# Autodesk Inventor assembly: BoronHead
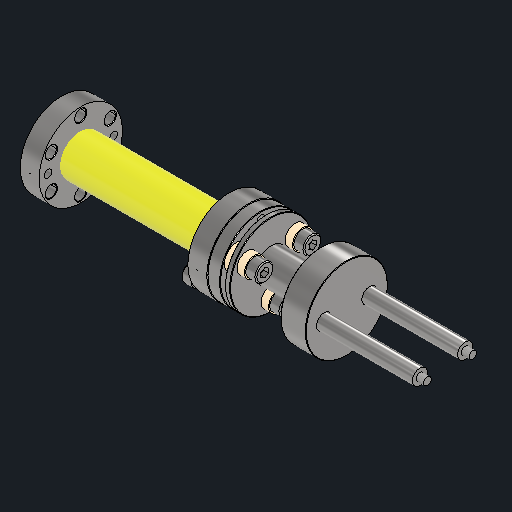
[picture p0: Inventor's stored thumbnail of the model, 512x512]
Saved by Autodesk Inventor 2027.1 (Build 311270010, 270A)
## iProperties
Created: 2025-06-19
Part Number: BoronHead
Document SubType Name: Assembly
Designer: kuzmin
Author: kuzmin
## Documents named in this file (8)
- C:\Users\queezz\Dropbox\Drawings\pihti-cad\BoronProbe\BoronHead.iam
- C:\Users\queezz\Dropbox\Drawings\pihti-cad\BoronProbe\HayashiProbeHead.ipt
- C:\Users\queezz\Dropbox\Drawings\pihti-cad\ContentCenter\Fastners\M4x10-SHCS.ipt
- C:\Users\queezz\Dropbox\Drawings\pihti-cad\BoronProbe\Shaft.ipt
- C:\Users\queezz\Dropbox\Drawings\pihti-cad\ContentCenter\Ceramics\ceramic_bushing_M4.ipt
- C:\Users\queezz\Dropbox\Drawings\pihti-cad\ContentCenter\Ceramics\ceramic_washer_M4.ipt
- C:\Users\queezz\Dropbox\Drawings\pihti-cad\PALP\CF34-nipples-for-PALP\ICF34_70mmNipple.iam
- C:\Users\queezz\Dropbox\Drawings\pihti-cad\BoronProbe\flange-adapter.ipt
## Components (16 placed, 7 different names)
1. HayashiProbeHead:1 — Rigid:4, Rigid:5, Rigid:6, Rotational:1, Rotational:2, Rigid:7, Rigid:8, Rigid:9, Mate:1, Mate:2
2. Shaft:1 — Rigid:5
3. Shaft:2 — Rigid:4
4. ceramic_bushing_M4:1 — Rigid:6, Rotational:5
5. ceramic_bushing_M4:2 — Rotational:1, Rotational:4
6. ceramic_bushing_M4:3 — Rotational:2, Rotational:3
7. ceramic_washer_M4:1 — Rigid:7
8. ceramic_washer_M4:2 — Rigid:8
9. ceramic_washer_M4:3 — Rigid:9, Mate:4
10. ICF34_70mmNipple:1 [sub-assembly] — Mate:1, Rigid:10, Rigid:11, Rotational:6
11. flange-adapter:1 — Mate:2, Mate:3, Mate:4, Rigid:10
12. AS 1420 - Metric M4 x 10:4 — Rigid:11
13. AS 1420 - Metric M4 x 10:5 — Rotational:6
14. AS 1420 - Metric M4 x 10:1 — Rotational:4
15. AS 1420 - Metric M4 x 10:2 — Rotational:5, Mate:3
16. AS 1420 - Metric M4 x 10:3 — Rotational:3
## Relationships (18: WeldJoint 8, RevoluteJoint 6, Mate 4)
- Rigid:4 [WeldJoint]: HayashiProbeHead:1 ↔ Shaft:2
- Rigid:5 [WeldJoint]: HayashiProbeHead:1 ↔ Shaft:1
- Rigid:6 [WeldJoint]: HayashiProbeHead:1 ↔ ceramic_bushing_M4:1
- Rotational:1 [RevoluteJoint]: HayashiProbeHead:1 ↔ ceramic_bushing_M4:2
- Rotational:2 [RevoluteJoint]: HayashiProbeHead:1 ↔ ceramic_bushing_M4:3
- Rotational:3 [RevoluteJoint]: ceramic_bushing_M4:3 ↔ AS 1420 - Metric M4 x 10:3
- Rotational:4 [RevoluteJoint]: ceramic_bushing_M4:2 ↔ AS 1420 - Metric M4 x 10:1
- Rotational:5 [RevoluteJoint]: ceramic_bushing_M4:1 ↔ AS 1420 - Metric M4 x 10:2
- Rigid:7 [WeldJoint]: HayashiProbeHead:1 ↔ ceramic_washer_M4:1
- Rigid:8 [WeldJoint]: HayashiProbeHead:1 ↔ ceramic_washer_M4:2
- Rigid:9 [WeldJoint]: HayashiProbeHead:1 ↔ ceramic_washer_M4:3
- Mate:1: HayashiProbeHead:1 ↔ ICF34_70mmNipple:1
- Mate:2: HayashiProbeHead:1 ↔ flange-adapter:1
- Mate:3: flange-adapter:1 ↔ AS 1420 - Metric M4 x 10:2
- Mate:4: ceramic_washer_M4:3 ↔ flange-adapter:1
- Rigid:10 [WeldJoint]: ICF34_70mmNipple:1 ↔ flange-adapter:1
- Rigid:11 [WeldJoint]: ICF34_70mmNipple:1 ↔ AS 1420 - Metric M4 x 10:4
- Rotational:6 [RevoluteJoint]: ICF34_70mmNipple:1 ↔ AS 1420 - Metric M4 x 10:5
